# Autodesk Inventor assembly: gears-smol-stack
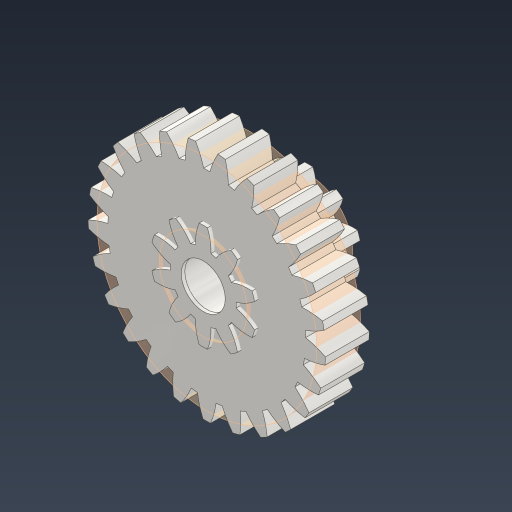
[picture p0: Inventor's stored thumbnail of the model, 512x512]
Saved by Autodesk Inventor 2023 (Build 270158000, 158)
## iProperties
Created: 2025-04-27
Part Number: gears-smol-stack
Document SubType Name: Assembly
Designer: szymo
Mass: 3 g
Surface Area: 7.16966 cm^2
Volume: 0.380623 cm^3
Author: szymo
## Documents named in this file (3)
- D:\tech\robotyka\robots\evangelion\inventor-project\gear-stack-small.iam
- D:\tech\robotyka\robots\evangelion\inventor-project\gears-smol-stack\Design Accelerator\Spur Gears2.iam
- D:\tech\robotyka\robots\evangelion\inventor-project\gears-smol-stack\Design Accelerator\Spur Gears3.iam
## Components (2 placed, 1 different names)
1. Spur Gears:1 [sub-assembly] — Flush:1, Mate:1, Mate:2
2. Spur Gears:2 [sub-assembly] — Flush:1, Mate:1, Mate:2
## Relationships (3: Mate 2, Flush 1)
- Flush:1 (0.2 mm): Spur Gears:1 ↔ Spur Gears:2
- Mate:1: Spur Gears:1 ↔ Spur Gears:2
- Mate:2: Spur Gears:1 ↔ Spur Gears:2
